# Autodesk Inventor assembly: Extruder
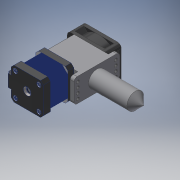
[picture p0: Inventor's stored thumbnail of the model, 180x180]
Saved by Autodesk Inventor 2019 (Build 230136000, 136)
## iProperties
Created: 2018-10-20
Part Number: Extruder
Document SubType Name: Assembly
Designer: LillaHunden
Author: LillaHunden
## Documents named in this file (4)
- C:\Users\LillaHunden\Documents\Inventor\3dprinter\3dPrinter\Extruder.iam
- C:\Users\LillaHunden\Documents\Inventor\3dprinter\3dPrinter\GT9S Extruder.ipt
- C:\Users\LillaHunden\Documents\Inventor\3dprinter\3dPrinter\Nema17 import\Nema 17HS4401-S.ipt
- C:\Users\LillaHunden\Documents\Inventor\3dprinter\3dPrinter\fan\GDSTIME 50mm x 50mm x 20mm 12V Brushless Cooling Fan.ipt
## Components (3 placed, 3 different names)
1. GT9S Extruder:1 — Mate:1, Angle:1, Flush:1, Flush:2, Mate:2, Flush:3
2. Nema 17HS4401-S:1 — Mate:1, Angle:1, Flush:1, Flush:2
3. GDSTIME 50mm x 50mm x 20mm 12V Brushless Cooling Fan:1 — Mate:2, Flush:3
## Relationships (6: Flush 3, Mate 2, Angle 1)
- Mate:1: GT9S Extruder:1 ↔ Nema 17HS4401-S:1
- Angle:1 (0 deg): GT9S Extruder:1 ↔ Nema 17HS4401-S:1
- Flush:1 (-2.5 mm): GT9S Extruder:1 ↔ Nema 17HS4401-S:1
- Flush:2 (-5.5 mm): GT9S Extruder:1 ↔ Nema 17HS4401-S:1
- Mate:2: GT9S Extruder:1 ↔ GDSTIME 50mm x 50mm x 20mm 12V Brushless Cooling Fan:1
- Flush:3: GT9S Extruder:1 ↔ GDSTIME 50mm x 50mm x 20mm 12V Brushless Cooling Fan:1
